# Autodesk Inventor assembly: sensor_placer
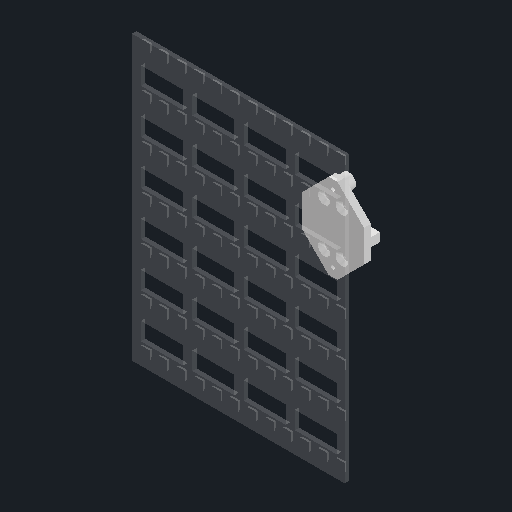
[picture p0: Inventor's stored thumbnail of the model, 512x512]
Saved by Autodesk Inventor 2026.1 (Build 301233000, 233)
## iProperties
Created: 2026-06-15
Part Number: sensor_placer
Document SubType Name: Assembly
Designer: aleja
Author: aleja
## Documents named in this file (3)
- C:\Users\aleja\Documents\iPV\Spatial_stability_3D_positioning\sensor_placer.iam
- C:\Users\aleja\Documents\iPV\Spatial_stability_3D_positioning\Platform.ipt
- C:\Users\aleja\Documents\iPV\Spatial_stability_3D_positioning\Base.ipt
## Components (2 placed, 2 different names)
1. Platform:1 — Mate:1, Flush:1, Flush:2
2. Base:1 — Mate:1, Flush:1, Flush:2
## Relationships (3: Flush 2, Mate 1)
- Mate:1 (1 mm): Platform:1 ↔ Base:1
- Flush:1 (-7.5 mm): Platform:1 ↔ Base:1
- Flush:2 (18 mm): Platform:1 ↔ Base:1
